# Autodesk Inventor assembly: AssembledOdourPort
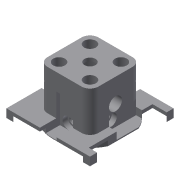
[picture p0: Inventor's stored thumbnail of the model, 180x180]
Saved by Autodesk Inventor 2018 (Build 220112000, 112)
## iProperties
Created: 2018-11-12
Part Number: AssembledOdourPort
Document SubType Name: Assembly
Designer: reinert
Author: reinert
## Documents named in this file (3)
- D:\PHD KUNER\#Paper_Beast\##SUPPLEMENT\CAD Files\OdourPort\AssembledOdourPort.iam
- D:\PHD KUNER\#Paper_Beast\##SUPPLEMENT\CAD Files\OdourPort\OdourPort_MainBody.ipt
- D:\PHD KUNER\#Paper_Beast\##SUPPLEMENT\CAD Files\OdourPort\OdourPort_Backplate.ipt
## Components (2 placed, 2 different names)
1. OdourPort_MainBody:1 — Mate:1, Flush:1, Flush:2
2. OdourPort_Backplate:1 — Mate:1, Flush:1, Flush:2
## Relationships (3: Flush 2, Mate 1)
- Mate:1: OdourPort_MainBody:1 ↔ OdourPort_Backplate:1
- Flush:1: OdourPort_MainBody:1 ↔ OdourPort_Backplate:1
- Flush:2: OdourPort_MainBody:1 ↔ OdourPort_Backplate:1
